# Autodesk Inventor assembly: coffeeShop
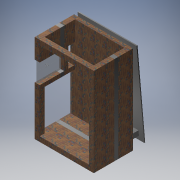
[picture p0: Inventor's stored thumbnail of the model, 180x180]
Saved by Autodesk Inventor 2019 (Build 230136000, 136)
## iProperties
Created: 2018-09-20
Part Number: coffeeShop
Document SubType Name: Assembly
Designer: wade
Author: wade
## Documents named in this file (5)
- C:\Users\wade\Documents\GitHub\UvicVRCityCAD\coffeeShop.iam
- C:\Users\wade\Documents\GitHub\UvicVRCityCAD\coffeeShopFrame.ipt
- C:\Users\wade\Documents\GitHub\UvicVRCityCAD\coffeeWindowFrontLeft.ipt
- C:\Users\wade\Documents\GitHub\UvicVRCityCAD\doorLeft.ipt
- C:\Users\wade\Documents\GitHub\UvicVRCityCAD\doorRight.ipt
## Components (4 placed, 4 different names)
1. coffeeShopFrame:1 — Mate:1, Mate:2, Mate:3, Mate:9, Mate:10, Mate:15, Mate:16, Flush:1, Mate:19, Mate:20, Flush:3, Mate:21, Mate:22, Flush:4
2. coffeeWindowFrontLeft:4 — Mate:15, Mate:16, Flush:1
3. doorLeft:1 — Mate:19, Mate:20, Flush:3
4. doorRight:1 — Mate:21, Mate:22, Flush:4
## Relationships (15: Mate 12, Flush 3)
- Mate:1: coffeeShopFrame:1
- Mate:2: coffeeShopFrame:1
- Mate:3: coffeeShopFrame:1
- Mate:9: coffeeShopFrame:1
- Mate:10: coffeeShopFrame:1
- Mate:14
- Mate:15: coffeeShopFrame:1 ↔ coffeeWindowFrontLeft:4
- Mate:16: coffeeShopFrame:1 ↔ coffeeWindowFrontLeft:4
- Flush:1 (166.6667 mm): coffeeShopFrame:1 ↔ coffeeWindowFrontLeft:4
- Mate:19: coffeeShopFrame:1 ↔ doorLeft:1
- Mate:20: coffeeShopFrame:1 ↔ doorLeft:1
- Flush:3 (166.6667 mm): coffeeShopFrame:1 ↔ doorLeft:1
- Mate:21: coffeeShopFrame:1 ↔ doorRight:1
- Mate:22: coffeeShopFrame:1 ↔ doorRight:1
- Flush:4 (166.6667 mm): coffeeShopFrame:1 ↔ doorRight:1
